# Autodesk Inventor assembly: CJ2D16-25Z(0_1)
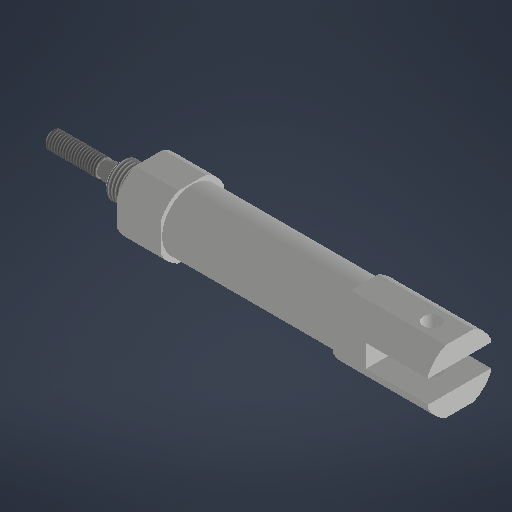
[picture p0: Inventor's stored thumbnail of the model, 512x512]
Saved by Autodesk Inventor 2025.2 (Build 292293000, 293)
## iProperties
Category: PARTsolutions
Company: SMC
Created: 2025-12-04
Part Number: CJ2D16-25Z(0_1)
Catalog Web Link: www.3dfindit.com
Description: CJ2-Z/CDJ2-Z-Air Cylinder/Standard: Double Acting Single Rod
Vendor: SMC
Document SubType Name: Assembly
Designer: psAdmin
Manufacturer: SMC
Mass: 18.3815 g
Surface Area: 116.655 cm^2
Volume: 18.3815 cm^3
Density: 1 g/cm^3
PSOL_IDENT_0: {$CADENAS_DATA/23d-libs/smc_jp/actuator/standard_air_cylinder/cj2/cj2_z_asmtab.prj},300 {VTYP=3D},{S
PSOL_IDENT_1: TYP=ASSTAB},{NB=CJ2D16-25Z(0_1)},{LINA=CJ2D16-25Z},{NN=CJ2-Z/CDJ2-Z},{DATE=21.08.2025 09:02:40},{GEO
PSOL_IDENT_2: MDATE=08.08.2025 00:20:55},{VERSION=},{LINEID=430},{WBVAR=MAGNET,AUTOSWITCH,LEAD,NUMBER,CUSHION,STRO
PSOL_IDENT_3: KE,POS,PORT,BRACKET,RODB,MOUNTING,OMSC,OMSCXC3,OMSCXC51,THREAD},{WBNUMERIC=STROKE,POS}  {NB=CJ2D16-2
PSOL_IDENT_4: 5Z(0_1)},{LINA=CJ2D16-25Z},{KT=DUMMY},{NENN=CJ2D16-25Z},{ORDER=CJ2D16-25Z},{BORE=16},{MOUNT=(D) Doub
PSOL_IDENT_5: le clevis},{MOUNTX=D},{MAGNET=},{AUTOSWITCH=},{AUTOSWX='','N/A'},{LEAD=},{LEADX= '','N/A' },{NUMBER=
PSOL_IDENT_6: },{CUSHION=},{CUSHIONX= '','(-) Rubber cushion','A','(A) Air cushion' },{SWSIGNX= '','N/A' },{STROKE=
PSOL_IDENT_7: 25},{COM=Please confirm the conditions of use with SMC},{STDSTROKE=15,30,45,60,75,100,125,150,175,20
PSOL_IDENT_8: 0},{STROKE1X=<20>,[1:400/1]},{SMIN=1},{SMINASW1=10},{SMINASW2=15},{SMAX1=400},{POS=0},{PORT=},{COM1=
PSOL_IDENT_9: -},{BRACKET=},{RODB=},{RODBX= '', '(-) None', 'V', '(V) Single knuckle joint', 'W'  , '(W) Double kn
PSOL_IDENT_10: uckle joint', 'T', '(T) Rod end cap (Flat type)', 'U'  , '(U) Rod end cap (Round type)' },{MOUNTING=
PSOL_IDENT_11: },{OMSC=},{OMSCXC3=},{OMSCXC51=},{THREAD=1},{MOUNTINGX='','N/A'},{BRACKETX='','(-) None','N','(N) Pi
PSOL_IDENT_12: vot bracket is shipped together with the product,but not assembled.'},{PORTX='', '(-) Perpendicular
PSOL_IDENT_13: to axis'},{SW=B},{OMSCX= '','(-) None','-XB6','(XB6) Heat resistant cylinder (-10 to 150 degree Cels
PSOL_IDENT_14: ius)','-XB7','(XB7) Cold resistant cylinder (-40 to 70 degree Celsius)','-XB9','(XB9) Low speed cyli
PSOL_IDENT_15: nder (10 to 50 mm/s)','-XC22','(XC22) Fluororubber seals','-XC85','(XC85) Grease specification for f
PSOL_IDENT_16: ood processing machines', '-X446'  , '(X446) PTFE grease' },{A=2.5},{XC3= '','(-) None','-XC3AB','(X
PSOL_IDENT_17: C3AB) Rod port location viewed: A,Head port location viewed: B','-XC3AC','(XC3AC) Rod port location
PSOL_IDENT_18: viewed: A,Head port location viewed: C','-XC3AD','(XC3AD) Rod port location viewed: A,Head port loca
PSOL_IDENT_19: tion viewed: D','-XC3BA','(XC3BA) Rod port location viewed: B,Head port location viewed: A','-XC3BB'
PSOL_IDENT_20: ,'(XC3BB) Rod port location viewed: B,Head port location viewed: B','-XC3BC','(XC3BC) Rod port locat
PSOL_IDENT_21: ion viewed: B,Head port location viewed: C','-XC3BD','(XC3BD) Rod port location viewed: B,Head port
PSOL_IDENT_22: location viewed: D','-XC3CA','(XC3CA) Rod port location viewed: C,Head port location viewed: A','-XC
PSOL_IDENT_23: 3CB','(XC3CB) Rod port location viewed: C,Head port location viewed: B','-XC3CC','(XC3CC) Rod port l
PSOL_IDENT_24: ocation viewed: C,Head port location viewed: C','-XC3CD','(XC3CD) Rod port location viewed: C,Head p
PSOL_IDENT_25: ort location viewed: D','-XC3DA','(XC3DA) Rod port location viewed: D,Head port location viewed: A','
PSOL_IDENT_26: -XC3DB','(XC3DB) Rod port location viewed: D,Head port location viewed: B','-XC3DC','(XC3DC) Rod por
PSOL_IDENT_27: t location viewed: D,Head port location viewed: C','-XC3DD','(XC3DD) Rod port location viewed: D,Hea
PSOL_IDENT_28: d port location viewed: D' },{XC51= '','(-) None','-XC51H4','(XC51H4) Hose nipple type: ø4/2.5 with
PSOL_IDENT_29: restriction','-XC51H6','(XC51H6) Hose nipple type: ø6/4 with restriction','-XC51MH4','(XC51MH4) Hose
PSOL_IDENT_30: nipple type: ø4/2.5 without restriction','-XC51MH6','(XC51MH6) Hose nipple type: ø6/4 without restr
PSOL_IDENT_31: iction' },{BMP=D},{PPATH=cj2_z/assembly/cj2_z_asmsbl.prj},{OMSCXX= '','(-) None','-XB6','(XB6) Heat
PSOL_IDENT_32: resistant cylinder (-10 to 150 degree Celsius)','-XB7','(XB7) Cold resistant cylinder (-40 to 70 deg
PSOL_IDENT_33: ree Celsius)','-XB9','(XB9) Low speed cylinder (10 to 50 mm/s)','-XC22','(XC22) Fluororubber seals','
PSOL_IDENT_34: -XC85','(XC85) Grease specification for food processing machines', '-X446' , '(X446) PTFE grease' ,'
PSOL_IDENT_35: -X2838','(X2838) Double clevis (With one-touch connecting pin)' }
NB: CJ2D16-25Z(0_1)
NN: CJ2-Z/CDJ2-Z
NT: Air Cylinder/Standard: Double Acting Single Rod
NBSYN: $ORDER.($POS._$THREAD.)
LINA: CJ2D16-25Z
CATALOG: SMC (JP
BORE: 16
MOUNT: (D) Double clevis
MAGNET: (-) Without magnet
AUTOSWITCH: N/A
LEAD: N/A
NUMBER: N/A
CUSHION: (-) Rubber cushion
STROKE: 25
POS: 0
PORT: (-) Perpendicular to axis
COM1: -
BRACKET: (-) None
RODB: (-) None
MOUNTING: N/A
OMSC: (-) None
OMSCXC3: (-) None
OMSCXC51: (-) None
THREAD: off
SUPPLIER: SMC
ARTICLENO: CJ2D16-25Z(0_1)
BOMINFO: CJ2D16-25Z
CREATOR: CADENAS GmbH
Title: CJ2D16-25Z
Author: Cadenas PARTsolutions
Comments: Air Cylinder/Standard: Double Acting Single Rod
## Documents named in this file (3)
- C:\Users\cloudy\Documents\GitHub\aura-cad\15\25 stroke 16 bore piston\CJ2D16-25Z(0_1).iam
- C:\Users\cloudy\Documents\GitHub\aura-cad\15\25 stroke 16 bore piston\CJ2D16-25Z(1_1)_BODY.ipt
- C:\Users\cloudy\Documents\GitHub\aura-cad\15\25 stroke 16 bore piston\CJ2D16-25Z_ROD.ipt
## Components (2 placed, 2 different names)
1. CJ2D16-25Z(1_1)_BODY:1 — Insert:1
2. CJ2D16-25Z_ROD:1 — Insert:1
## Relationships (1: Insert 1)
- Insert:1: CJ2D16-25Z(1_1)_BODY:1 ↔ CJ2D16-25Z_ROD:1
